# Autodesk Inventor assembly: Perfil-de-aluminio-0001-001
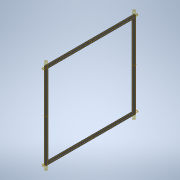
[picture p0: Inventor's stored thumbnail of the model, 180x180]
Saved by Autodesk Inventor 2020.1 (Build 241239000, 239)
## iProperties
Created: 2024-04-06
Part Number: Perfil-de-aluminio-0001-001
Document SubType Name: Assembly
Designer: MiguelBarbosa
Author: MiguelBarbosa
## Documents named in this file (2)
- D:\Portugal\IEFP_Porto\Presente\6415_Desenho_de_construcao_mecanica\6415_Construcao_Mecanica\Sessoes\Sessao4\Perfil-de-aluminio-0001-001.iam
- D:\Portugal\IEFP_Porto\Presente\6415_Desenho_de_construcao_mecanica\6415_Construcao_Mecanica\Sessoes\Sessao4\Perfil-de-aluminio-0001-001.ipt
## Components (4 placed, 1 different names)
1. Perfil-de-aluminio-0001-001:1 — Flush:1, Flush:2, Flush:3, Flush:7, Mate:1
2. Perfil-de-aluminio-0001-001:2 — Flush:1, Flush:2, Flush:6, Mate:2, Flush:8
3. Perfil-de-aluminio-0001-001:3 — Flush:3, Flush:4, Flush:5, Flush:8
4. Perfil-de-aluminio-0001-001:4 — Flush:5, Flush:6, Flush:7, Mate:1, Mate:2
## Relationships (10: Flush 8, Mate 2)
- Flush:1: Perfil-de-aluminio-0001-001:1 ↔ Perfil-de-aluminio-0001-001:2
- Flush:2: Perfil-de-aluminio-0001-001:1 ↔ Perfil-de-aluminio-0001-001:2
- Flush:3: Perfil-de-aluminio-0001-001:1 ↔ Perfil-de-aluminio-0001-001:3
- Flush:4: Perfil-de-aluminio-0001-001:3
- Flush:5: Perfil-de-aluminio-0001-001:3 ↔ Perfil-de-aluminio-0001-001:4
- Flush:6: Perfil-de-aluminio-0001-001:2 ↔ Perfil-de-aluminio-0001-001:4
- Flush:7: Perfil-de-aluminio-0001-001:1 ↔ Perfil-de-aluminio-0001-001:4
- Mate:1: Perfil-de-aluminio-0001-001:1 ↔ Perfil-de-aluminio-0001-001:4
- Mate:2: Perfil-de-aluminio-0001-001:2 ↔ Perfil-de-aluminio-0001-001:4
- Flush:8: Perfil-de-aluminio-0001-001:2 ↔ Perfil-de-aluminio-0001-001:3
